# Autodesk Inventor assembly: plate
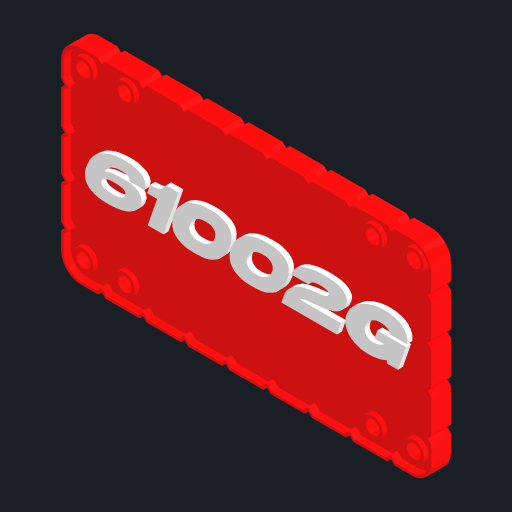
[picture p0: Inventor's stored thumbnail of the model, 512x512]
Saved by Autodesk Inventor 2024.2 (Build 282272000, 272)
## iProperties
Created: 2024-01-31
Part Number: plate
Document SubType Name: Assembly
Designer: reima
Author: reima
## Documents named in this file (3)
- O:\cad\61002g-cad\VEX parts\Miscellaneous\plate.iam
- O:\cad\61002g-cad\VEX parts\Miscellaneous\Red License Plate.ipt
- O:\cad\61002g-cad\VEX parts\Miscellaneous\name v1.ipt
## Components (2 placed, 2 different names)
1. Red License Plate:1 — Mate:1
2. name v1:1 — Mate:1
## Relationships (1: Mate 1)
- Mate:1: Red License Plate:1 ↔ name v1:1
